# Autodesk Inventor assembly: spherical manipulator base
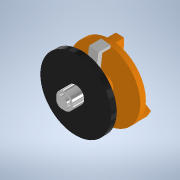
[picture p0: Inventor's stored thumbnail of the model, 180x180]
Saved by Autodesk Inventor 2021 (Build 250183000, 183)
## iProperties
Created: 2021-05-05
Part Number: spherical manipulator base
Document SubType Name: Assembly
Designer: techv
Author: techv
## Documents named in this file (7)
- D:\Projects\P_Borewell\V2\Design\spherical manipulator base.iam
- D:\Projects\P_Borewell\V2\Design\PM Base.ipt
- D:\Projects\P_Borewell\V2\Design\lead_screw.ipt
- D:\Projects\P_Borewell\V2\Design\Bot Base.ipt
- D:\Projects\P_Borewell\V2\Design\Motor.ipt
- D:\Projects\P_Borewell\V2\Design\z axis base.ipt
- D:\Projects\P_Borewell\V2\Design\pm connector.ipt
## Components (6 placed, 6 different names)
1. PM Base:1 — Mate:5, Mate:6, Mate:8
2. lead_screw:1 — Mate:4, Flush:2, Mate:7
3. Bot Base:1 — Mate:1, Flush:1, Flush:3
4. Motor:1 — Mate:1, Flush:1, Mate:2, Mate:3
5. z axis base:1 — Mate:2, Mate:3, Mate:4, Flush:2
6. pm connector:1 — Mate:5, Mate:6, Mate:7
## Relationships (11: Mate 8, Flush 3)
- Mate:1: Bot Base:1 ↔ Motor:1
- Flush:1: Bot Base:1 ↔ Motor:1
- Mate:2: Motor:1 ↔ z axis base:1
- Mate:3: Motor:1 ↔ z axis base:1
- Mate:4: lead_screw:1 ↔ z axis base:1
- Flush:2: lead_screw:1 ↔ z axis base:1
- Mate:5: PM Base:1 ↔ pm connector:1
- Mate:6: PM Base:1 ↔ pm connector:1
- Mate:7: lead_screw:1 ↔ pm connector:1
- Flush:3 (43.5 mm): Bot Base:1
- Mate:8: PM Base:1
